# Autodesk Inventor assembly: Roll
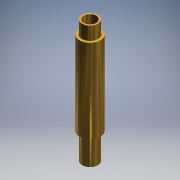
[picture p0: Inventor's stored thumbnail of the model, 180x180]
Saved by Autodesk Inventor 2018.3 (Build 223284000, 284)
## iProperties
Created: 2018-08-03
Part Number: Roll
Material: Generisch
Document SubType Name: Assembly
Designer: JochenAlt
Author: JochenAlt
## Documents named in this file (3)
- D:\Projects\FlowerPot\CAD\CycloidalGear2\Roll.iam
- D:\Projects\FlowerPot\CAD\CycloidalGear2\Rolls.ipt
- D:\Projects\FlowerPot\CAD\CycloidalGear2\RollAxis.ipt
## Components (2 placed, 2 different names)
1. Rolls:1 — Passend:1, 2
2. RollAxis:1 — Passend:1, 2
## Relationships (2: Mate 1, Flush 1)
- Passend:1 [Mate]: Rolls:1 ↔ RollAxis:1
- 2 [Flush] (2.5 mm): Rolls:1 ↔ RollAxis:1
